# Autodesk Inventor assembly: 2020Robot
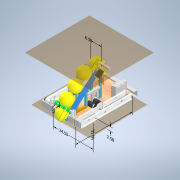
[picture p0: Inventor's stored thumbnail of the model, 180x180]
Saved by Autodesk Inventor 2022.1 (Build 261234020, 234B)
## iProperties
Created: 2020-01-25
Part Number: 2020Robot
Document SubType Name: Assembly
Designer: robst
Author: robst
## Documents named in this file (19)
- C:\git\CAD-Development\robSteele\2020CompetitionRobot\2020Robot.iam
- C:\git\CAD-Development\robSteele\2020CompetitionRobot\woodBase.ipt
- C:\git\CAD-Development\robSteele\2020CompetitionRobot\ballRampWithStepForBallLeftSide.iam
- C:\git\CAD-Development\robSteele\2020CompetitionRobot\ballRampWithStepForBallRightSide.iam
- C:\git\CAD-Development\robSteele\2020CompetitionRobot\am-3312a_Gear Intake Kit Gear Config.iam
- C:\git\CAD-Development\robSteele\2020CompetitionRobot\am-3922 AM14U4 Inside Plate.ipt
- C:\git\CAD-Development\robSteele\2020CompetitionRobot\am-3921 AM14U4 Outside Plate.ipt
- C:\git\CAD-Development\robSteele\2020CompetitionRobot\am-3922 AM14U4 Inside Plate_MIR.ipt
- C:\git\CAD-Development\robSteele\2020CompetitionRobot\am-3921 AM14U4 Outside Plate_MIR.ipt
- C:\git\CAD-Development\robSteele\2020CompetitionRobot\2020 End Plate.ipt
- C:\git\CAD-Development\robSteele\2020CompetitionRobot\2020 Front Plate.ipt
- C:\git\CAD-Development\robSteele\2020CompetitionRobot\2020 Front Plate_MIR.ipt
- C:\git\CAD-Development\robSteele\2020CompetitionRobot\ToughBoxMiniWith2CimMotors.iam
- C:\git\CAD-Development\robSteele\2020CompetitionRobot\ToughBoxMiniWith2CimMotors_MIR.iam
- C:\git\CAD-Development\robSteele\2020CompetitionRobot\1892-YEL.ipt
- C:\git\CAD-Development\robSteele\2020CompetitionRobot\shooter.iam
- C:\git\CAD-Development\robSteele\2020LongRobotBase\floor.ipt
- C:\git\CAD-Development\robSteele\2020CompetitionRobot\ceiling.ipt
- C:\git\CAD-Development\robSteele\2020CompetitionRobot\battery.ipt
## Components (22 placed, 18 different names)
1. woodBase:1 — Flush:1, Flush:2, Flush:3, Mate:1, Mate:4, Mate:7, Flush:5, Mate:8, Mate:9, Mate:13, Mate:14, Mate:15, Mate:16, Mate:31, Mate:45
2. ballRampWithStepForBallLeftSide:1 [sub-assembly] — Mate:1, Mate:3, Mate:28, Mate:29, Mate:38, Mate:30, Mate:42, Mate:43, Mate:44, Tangent:5
3. ballRampWithStepForBallRightSide:1 [sub-assembly] — Mate:4, Flush:4
4. am-3312a_Gear Intake Kit Gear Config:1 [sub-assembly] — Mate:6, Mate:7, Flush:5
5. am-3922 AM14U4 Inside Plate:1 — Mate:8, Flush:10, Mate:9, Flush:11, Flush:12, Mate:10, Insert:1, Insert:2, Mate:47
6. am-3921 AM14U4 Outside Plate:1 — Flush:11, Flush:12, Mate:10, Flush:16
7. am-3922 AM14U4 Inside Plate_MIR:1 — Mate:11, Mate:12, Flush:13, Flush:14
8. am-3921 AM14U4 Outside Plate_MIR:1 — Mate:12, Flush:13, Flush:14
9. 2020 End Plate:1 — Flush:15, Mate:13, Mate:14, Mate:46
10. 2020 Front Plate:1 — Mate:15, Mate:16, Flush:16
11. 2020 Front Plate_MIR:1
12. ToughBoxMiniWith2CimMotors:1 [sub-assembly] — Insert:1, Insert:2, Tangent:5
13. ToughBoxMiniWith2CimMotors_MIR:1 [sub-assembly]
14. 1892-YEL:1 — Mate:27, Mate:28, Mate:29
15. shooter:1 [sub-assembly] — Mate:38, Mate:30
16. floor:1 — Mate:31, Mate:32, Mate:33, Mate:34, Tangent:1
17. ceiling:1 — Mate:34, Mate:35, Mate:36
18. 1892-YEL:2 — Mate:37, Tangent:1, Tangent:2
19. 1892-YEL:3 — Mate:39, Mate:42, Tangent:2, Tangent:3
20. 1892-YEL:4 — Mate:40, Mate:43, Tangent:3, Tangent:4
21. 1892-YEL:5 — Mate:41, Mate:44, Tangent:4
22. battery:1 — Mate:45, Mate:46, Mate:47
## Relationships (54: Mate 35, Flush 12, Tangent 5, Insert 2)
- Flush:1: woodBase:1
- Flush:2: woodBase:1
- Flush:3: woodBase:1
- Mate:1: woodBase:1 ↔ ballRampWithStepForBallLeftSide:1
- Mate:3 (57.15 mm): ballRampWithStepForBallLeftSide:1
- Mate:4: woodBase:1 ↔ ballRampWithStepForBallRightSide:1
- Flush:4 (-57.15 mm): ballRampWithStepForBallRightSide:1
- Mate:6: am-3312a_Gear Intake Kit Gear Config:1
- Mate:7 (12.7 mm): woodBase:1 ↔ am-3312a_Gear Intake Kit Gear Config:1
- Flush:5: woodBase:1 ↔ am-3312a_Gear Intake Kit Gear Config:1
- Mate:8: woodBase:1 ↔ am-3922 AM14U4 Inside Plate:1
- Flush:10: am-3922 AM14U4 Inside Plate:1
- Mate:9: woodBase:1 ↔ am-3922 AM14U4 Inside Plate:1
- Flush:11: am-3922 AM14U4 Inside Plate:1 ↔ am-3921 AM14U4 Outside Plate:1
- Flush:12: am-3922 AM14U4 Inside Plate:1 ↔ am-3921 AM14U4 Outside Plate:1
- Mate:10 (85.725 mm): am-3922 AM14U4 Inside Plate:1 ↔ am-3921 AM14U4 Outside Plate:1
- Mate:11: am-3922 AM14U4 Inside Plate_MIR:1
- Mate:12 (85.725 mm): am-3922 AM14U4 Inside Plate_MIR:1 ↔ am-3921 AM14U4 Outside Plate_MIR:1
- Flush:13: am-3922 AM14U4 Inside Plate_MIR:1 ↔ am-3921 AM14U4 Outside Plate_MIR:1
- Flush:14: am-3922 AM14U4 Inside Plate_MIR:1 ↔ am-3921 AM14U4 Outside Plate_MIR:1
- Flush:15: 2020 End Plate:1
- Mate:13: woodBase:1 ↔ 2020 End Plate:1
- Mate:14: woodBase:1 ↔ 2020 End Plate:1
- Mate:15: woodBase:1 ↔ 2020 Front Plate:1
- Mate:16: woodBase:1 ↔ 2020 Front Plate:1
- Flush:16: am-3921 AM14U4 Outside Plate:1 ↔ 2020 Front Plate:1
- Insert:1: am-3922 AM14U4 Inside Plate:1 ↔ ToughBoxMiniWith2CimMotors:1
- Insert:2: am-3922 AM14U4 Inside Plate:1 ↔ ToughBoxMiniWith2CimMotors:1
- Mate:27: 1892-YEL:1
- Mate:28 (-25.4 mm): ballRampWithStepForBallLeftSide:1 ↔ 1892-YEL:1
- Mate:29 (-25.4 mm): ballRampWithStepForBallLeftSide:1 ↔ 1892-YEL:1
- Mate:38: ballRampWithStepForBallLeftSide:1 ↔ shooter:1
- Mate:30: ballRampWithStepForBallLeftSide:1 ↔ shooter:1
- Mate:31 (50.8 mm): woodBase:1 ↔ floor:1
- Mate:32: floor:1
- Mate:33: floor:1
- Mate:34 (711.2 mm): floor:1 ↔ ceiling:1
- Mate:35: ceiling:1
- Mate:36: ceiling:1
- Mate:37: 1892-YEL:2
- Tangent:1: floor:1 ↔ 1892-YEL:2
- Mate:39: 1892-YEL:3
- Mate:40: 1892-YEL:4
- Mate:41: 1892-YEL:5
- Mate:42: ballRampWithStepForBallLeftSide:1 ↔ 1892-YEL:3
- Tangent:2: 1892-YEL:2 ↔ 1892-YEL:3
- Mate:43: ballRampWithStepForBallLeftSide:1 ↔ 1892-YEL:4
- Tangent:3: 1892-YEL:3 ↔ 1892-YEL:4
- Mate:44: ballRampWithStepForBallLeftSide:1 ↔ 1892-YEL:5
- Tangent:4: 1892-YEL:4 ↔ 1892-YEL:5
- Mate:45: woodBase:1 ↔ battery:1
- Mate:46: 2020 End Plate:1 ↔ battery:1
- Mate:47: am-3922 AM14U4 Inside Plate:1 ↔ battery:1
- Tangent:5: ballRampWithStepForBallLeftSide:1 ↔ ToughBoxMiniWith2CimMotors:1
